# Autodesk Inventor assembly: assembly_balancing
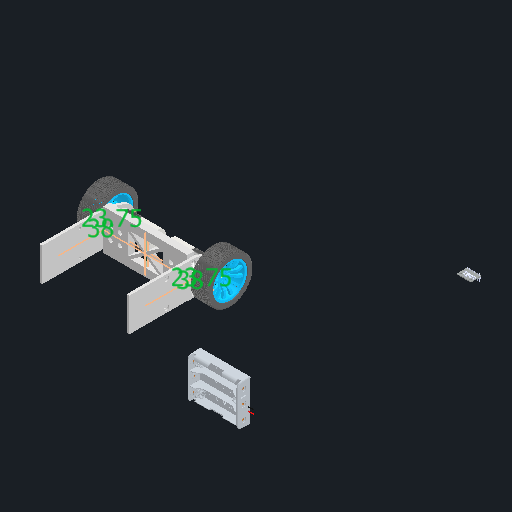
[picture p0: Inventor's stored thumbnail of the model, 512x512]
Saved by Autodesk Inventor 2026 (Build 300175000, 175)
## iProperties
Created: 2026-08-02
Part Number: assembly_balancing
Document SubType Name: Assembly
Designer: imcle
Author: imcle
## Documents named in this file (8)
- D:\Mechatronik\Prj\Self Balancing\assembly_balancing.iam
- D:\Mechatronik\Prj\Self Balancing\motor\25ga-370-280-rpm-dc Motor.ipt
- D:\Mechatronik\Prj\Self Balancing\do_ga'\do_ga.ipt
- D:\Mechatronik\Prj\Self Balancing\base\plate.ipt
- D:\Mechatronik\Prj\Self Balancing\65mm\蓝色轮胎\65mm蓝色轮胎总装-实际外径68mm\65mm蓝色轮胎总装-实际外径68mm\65mm蓝色轮胎总装-实际外径68mm.ipt
- D:\Mechatronik\Prj\Self Balancing\mpu6050\MPU6050\MPU6050\MPU6050.ipt
- D:\Mechatronik\Prj\Self Balancing\plate_base\plate_base.ipt
- D:\Mechatronik\Prj\Self Balancing\battery-case-for-3-18650-lion-1.snapshot.3\batteryCase18650x3\batteryCase18650x3\batteryCase18650x3.ipt
## Components (11 placed, 7 different names)
1. 25ga-370-280-rpm-dc Motor:1 — Rigid:1, Rotational:1
2. 25ga-370-280-rpm-dc Motor:2 — Rigid:2, Rotational:2
3. do_ga:1 — Rigid:1, Rigid:3, Rigid:5
4. do_ga:2 — Rigid:2, Rigid:4, Rigid:6
5. plate:2 — Rigid:3, Rigid:4, Mate:1
6. 65mm蓝色轮胎总装-实际外径68mm:1 — Rotational:1
7. 65mm蓝色轮胎总装-实际外径68mm:2 — Rotational:2
8. MPU6050:1
9. plate_base:1 — Rigid:5
10. plate_base:2 — Rigid:6
11. batteryCase18650x3:1 — Mate:1
## Relationships (9: WeldJoint 6, RevoluteJoint 2, Mate 1)
- Rigid:1 [WeldJoint]: 25ga-370-280-rpm-dc Motor:1 ↔ do_ga:1
- Rigid:2 [WeldJoint]: 25ga-370-280-rpm-dc Motor:2 ↔ do_ga:2
- Rigid:3 [WeldJoint]: do_ga:1 ↔ plate:2
- Rigid:4 [WeldJoint]: do_ga:2 ↔ plate:2
- Rotational:1 [RevoluteJoint]: 25ga-370-280-rpm-dc Motor:1 ↔ 65mm蓝色轮胎总装-实际外径68mm:1
- Rigid:5 [WeldJoint]: do_ga:1 ↔ plate_base:1
- Rigid:6 [WeldJoint]: do_ga:2 ↔ plate_base:2
- Rotational:2 [RevoluteJoint]: 25ga-370-280-rpm-dc Motor:2 ↔ 65mm蓝色轮胎总装-实际外径68mm:2
- Mate:1: plate:2 ↔ batteryCase18650x3:1
